# Autodesk Inventor assembly: main_pcb.brd
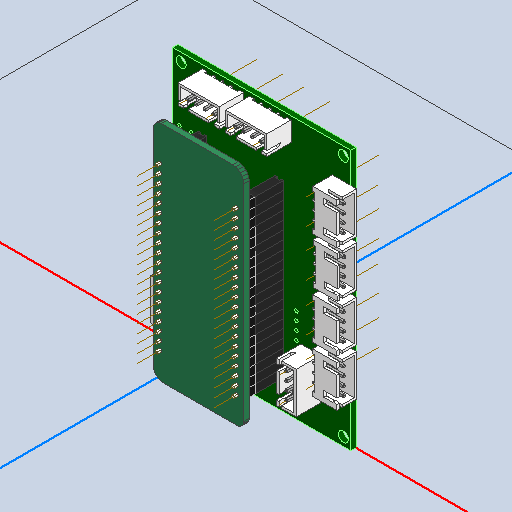
[picture p0: Inventor's stored thumbnail of the model, 512x512]
Saved by Autodesk Inventor 2022 (Build 260153000, 153)
## iProperties
Created: 2021-08-05
Part Number: main_pcb.brd
Document SubType Name: Assembly
Designer: Петров Иван
Mass: 18.6028 g
Surface Area: 275.031 cm^2
Volume: 13.5279 cm^3
Density: 1.37514 g/cm^3
Author: Петров Иван
## Documents named in this file (7)
- D:\IVAN\Ivan_desktop\Kvantorium\Projects\YouBotRobot\design\000.004 - Котроллер СНУ.iam
- D:\IVAN\Ivan_desktop\Kvantorium\Projects\YouBotRobot\design\standart_components\PBS-1.ipt
- D:\IVAN\Ivan_desktop\Kvantorium\Projects\YouBotRobot\design\standart_components\connectrs\JST - XH - Thru (R) - 4Pin - 2.54mm.ipt
- D:\IVAN\Ivan_desktop\Kvantorium\Projects\YouBotRobot\design\standart_components\connectrs\JST - XH - Thru (V) - 4Pin - 2.54mm.ipt
- D:\IVAN\Ivan_desktop\Kvantorium\Projects\YouBotRobot\design\000.004.001 - Плата печатная.ipt
- D:\IVAN\Ivan_desktop\Kvantorium\Projects\YouBotRobot\design\standart_components\CONN HEADER VERT 1POS 2.54MM.ipt
- D:\IVAN\Ivan_desktop\Kvantorium\Projects\YouBotRobot\design\standart_components\opencm904.ipt
## Components (90 placed, 6 different names)
1. 000.004.001 - Плата печатная.ipt:1 — Совмещение:15, Совмещение:16, Совмещение:17, Совмещение:18, Совмещение:19, Совмещение:20, Совмещение:26, Совмещение:27, Совмещение:28, Совмещение:29, Совмещение:30, Совмещение:31
2. JST - XH - Thru (R) - 4Pin - 2.54mm.ipt:1
3. JST - XH - Thru (R) - 4Pin - 2.54mm.ipt:2
4. JST - XH - Thru (V) - 4Pin - 2.54mm.ipt:1
5. JST - XH - Thru (V) - 4Pin - 2.54mm.ipt:2
6. JST - XH - Thru (R) - 4Pin - 2.54mm.ipt:3 — Совмещение:18, Совмещение:19, Совмещение:20
7. JST - XH - Thru (R) - 4Pin - 2.54mm.ipt:4 — Совмещение:15, Совмещение:16, Совмещение:17
8. opencm904.ipt:1 — Совмещение:23, Совмещение:24, Совмещение:25
9. JST - XH - Thru (V) - 4Pin - 2.54mm.ipt:3 — Совмещение:26, Совмещение:27, Совмещение:28
10. JST - XH - Thru (V) - 4Pin - 2.54mm.ipt:4 — Совмещение:29, Совмещение:30, Совмещение:31
11. PBS-1.ipt:1 — Совмещение:21, Совмещение:22, Заподлицо:1
12. PBS-1.ipt:2
13. PBS-1.ipt:3
14. PBS-1.ipt:4
15. PBS-1.ipt:5
16. PBS-1.ipt:6
17. PBS-1.ipt:7
18. PBS-1.ipt:8
19. PBS-1.ipt:9
20. PBS-1.ipt:10
21. PBS-1.ipt:11
22. PBS-1.ipt:12
23. PBS-1.ipt:13
24. PBS-1.ipt:14
25. PBS-1.ipt:15
26. PBS-1.ipt:16
27. PBS-1.ipt:17
28. PBS-1.ipt:18
29. PBS-1.ipt:19
30. PBS-1.ipt:20
31. PBS-1.ipt:21
32. PBS-1.ipt:22
33. PBS-1.ipt:23
34. PBS-1.ipt:24
35. PBS-1.ipt:25
36. PBS-1.ipt:26
37. PBS-1.ipt:27
38. PBS-1.ipt:28
39. PBS-1.ipt:29
40. PBS-1.ipt:30
41. PBS-1.ipt:31
42. PBS-1.ipt:32
43. PBS-1.ipt:33
44. PBS-1.ipt:34
45. PBS-1.ipt:35
46. PBS-1.ipt:36
47. PBS-1.ipt:37
48. PBS-1.ipt:38
49. PBS-1.ipt:39
50. PBS-1.ipt:40
51. CONN HEADER VERT 1POS 2.54MM.ipt:1 — Совмещение:21, Совмещение:22, Заподлицо:1, Совмещение:23, Совмещение:24
52. CONN HEADER VERT 1POS 2.54MM.ipt:2
53. CONN HEADER VERT 1POS 2.54MM.ipt:3
54. CONN HEADER VERT 1POS 2.54MM.ipt:4
55. CONN HEADER VERT 1POS 2.54MM.ipt:5
56. CONN HEADER VERT 1POS 2.54MM.ipt:6
57. CONN HEADER VERT 1POS 2.54MM.ipt:7
58. CONN HEADER VERT 1POS 2.54MM.ipt:8
59. CONN HEADER VERT 1POS 2.54MM.ipt:9
60. CONN HEADER VERT 1POS 2.54MM.ipt:10
61. CONN HEADER VERT 1POS 2.54MM.ipt:11
62. CONN HEADER VERT 1POS 2.54MM.ipt:12
63. CONN HEADER VERT 1POS 2.54MM.ipt:13
64. CONN HEADER VERT 1POS 2.54MM.ipt:14
65. CONN HEADER VERT 1POS 2.54MM.ipt:15
66. CONN HEADER VERT 1POS 2.54MM.ipt:16
67. CONN HEADER VERT 1POS 2.54MM.ipt:17
68. CONN HEADER VERT 1POS 2.54MM.ipt:18
69. CONN HEADER VERT 1POS 2.54MM.ipt:19
70. CONN HEADER VERT 1POS 2.54MM.ipt:20
71. CONN HEADER VERT 1POS 2.54MM.ipt:21
72. CONN HEADER VERT 1POS 2.54MM.ipt:22
73. CONN HEADER VERT 1POS 2.54MM.ipt:23
74. CONN HEADER VERT 1POS 2.54MM.ipt:24
75. CONN HEADER VERT 1POS 2.54MM.ipt:25
76. CONN HEADER VERT 1POS 2.54MM.ipt:26
77. CONN HEADER VERT 1POS 2.54MM.ipt:27
78. CONN HEADER VERT 1POS 2.54MM.ipt:28
79. CONN HEADER VERT 1POS 2.54MM.ipt:29
80. CONN HEADER VERT 1POS 2.54MM.ipt:30
81. CONN HEADER VERT 1POS 2.54MM.ipt:31
82. CONN HEADER VERT 1POS 2.54MM.ipt:32
83. CONN HEADER VERT 1POS 2.54MM.ipt:33
84. CONN HEADER VERT 1POS 2.54MM.ipt:34
85. CONN HEADER VERT 1POS 2.54MM.ipt:35
86. CONN HEADER VERT 1POS 2.54MM.ipt:36
87. CONN HEADER VERT 1POS 2.54MM.ipt:37
88. CONN HEADER VERT 1POS 2.54MM.ipt:38
89. CONN HEADER VERT 1POS 2.54MM.ipt:39
90. CONN HEADER VERT 1POS 2.54MM.ipt:40 — Совмещение:25
## Component patterns: (40 elements, first: PBS-1.ipt:1), (40 elements, first: CONN HEADER VERT 1POS 2.54MM.ipt:1)
## Relationships (33: Mate 31, Angle 1, Flush 1)
- [Mate]: 000.004.001 - Плата печатная.ipt:1 ↔ PBS-1.ipt:1
- [Angle] (90 deg): 000.004.001 - Плата печатная.ipt:1 ↔ PBS-1.ipt:1
- [Mate]: 000.004.001 - Плата печатная.ipt:1 ↔ PBS-1.ipt:1
- [Mate]: 000.004.001 - Плата печатная.ipt:1 ↔ JST - XH - Thru (R) - 4Pin - 2.54mm.ipt:1
- [Mate]: 000.004.001 - Плата печатная.ipt:1 ↔ JST - XH - Thru (R) - 4Pin - 2.54mm.ipt:1
- [Mate]: 000.004.001 - Плата печатная.ipt:1 ↔ JST - XH - Thru (R) - 4Pin - 2.54mm.ipt:1
- [Mate]: 000.004.001 - Плата печатная.ipt:1 ↔ JST - XH - Thru (R) - 4Pin - 2.54mm.ipt:2
- [Mate]: 000.004.001 - Плата печатная.ipt:1 ↔ JST - XH - Thru (R) - 4Pin - 2.54mm.ipt:2
- [Mate]: 000.004.001 - Плата печатная.ipt:1 ↔ JST - XH - Thru (R) - 4Pin - 2.54mm.ipt:2
- [Mate]: 000.004.001 - Плата печатная.ipt:1 ↔ JST - XH - Thru (V) - 4Pin - 2.54mm.ipt:1
- [Mate]: 000.004.001 - Плата печатная.ipt:1 ↔ JST - XH - Thru (V) - 4Pin - 2.54mm.ipt:1
- [Mate]: 000.004.001 - Плата печатная.ipt:1 ↔ JST - XH - Thru (V) - 4Pin - 2.54mm.ipt:1
- [Mate]: 000.004.001 - Плата печатная.ipt:1 ↔ JST - XH - Thru (V) - 4Pin - 2.54mm.ipt:2
- [Mate]: 000.004.001 - Плата печатная.ipt:1 ↔ JST - XH - Thru (V) - 4Pin - 2.54mm.ipt:2
- [Mate]: 000.004.001 - Плата печатная.ipt:1 ↔ JST - XH - Thru (V) - 4Pin - 2.54mm.ipt:2
- Совмещение:15 [Mate]: 000.004.001 - Плата печатная.ipt:1 ↔ JST - XH - Thru (R) - 4Pin - 2.54mm.ipt:4
- Совмещение:16 [Mate]: 000.004.001 - Плата печатная.ipt:1 ↔ JST - XH - Thru (R) - 4Pin - 2.54mm.ipt:4
- Совмещение:17 [Mate]: 000.004.001 - Плата печатная.ipt:1 ↔ JST - XH - Thru (R) - 4Pin - 2.54mm.ipt:4
- Совмещение:18 [Mate]: 000.004.001 - Плата печатная.ipt:1 ↔ JST - XH - Thru (R) - 4Pin - 2.54mm.ipt:3
- Совмещение:19 [Mate]: 000.004.001 - Плата печатная.ipt:1 ↔ JST - XH - Thru (R) - 4Pin - 2.54mm.ipt:3
- Совмещение:20 [Mate]: 000.004.001 - Плата печатная.ipt:1 ↔ JST - XH - Thru (R) - 4Pin - 2.54mm.ipt:3
- Совмещение:21 [Mate]: PBS-1.ipt:1 ↔ CONN HEADER VERT 1POS 2.54MM.ipt:1
- Совмещение:22 [Mate]: PBS-1.ipt:1 ↔ CONN HEADER VERT 1POS 2.54MM.ipt:1
- Заподлицо:1 [Flush]: PBS-1.ipt:1 ↔ CONN HEADER VERT 1POS 2.54MM.ipt:1
- Совмещение:23 [Mate]: opencm904.ipt:1 ↔ CONN HEADER VERT 1POS 2.54MM.ipt:1
- Совмещение:24 [Mate]: opencm904.ipt:1 ↔ CONN HEADER VERT 1POS 2.54MM.ipt:1
- Совмещение:25 [Mate]: opencm904.ipt:1 ↔ CONN HEADER VERT 1POS 2.54MM.ipt:40
- Совмещение:26 [Mate]: 000.004.001 - Плата печатная.ipt:1 ↔ JST - XH - Thru (V) - 4Pin - 2.54mm.ipt:3
- Совмещение:27 [Mate]: 000.004.001 - Плата печатная.ipt:1 ↔ JST - XH - Thru (V) - 4Pin - 2.54mm.ipt:3
- Совмещение:28 [Mate]: 000.004.001 - Плата печатная.ipt:1 ↔ JST - XH - Thru (V) - 4Pin - 2.54mm.ipt:3
- Совмещение:29 [Mate]: 000.004.001 - Плата печатная.ipt:1 ↔ JST - XH - Thru (V) - 4Pin - 2.54mm.ipt:4
- Совмещение:30 [Mate]: 000.004.001 - Плата печатная.ipt:1 ↔ JST - XH - Thru (V) - 4Pin - 2.54mm.ipt:4
- Совмещение:31 [Mate]: 000.004.001 - Плата печатная.ipt:1 ↔ JST - XH - Thru (V) - 4Pin - 2.54mm.ipt:4
